# Autodesk Inventor assembly: EEZYbotARM Mk2
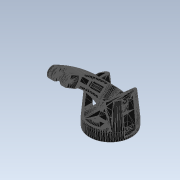
[picture p0: Inventor's stored thumbnail of the model, 180x180]
Saved by Autodesk Inventor 2022.5 (Build 265521000, 521)
## iProperties
Created: 2024-11-13
Part Number: EEZYbotARM Mk2
Document SubType Name: Assembly
Designer: Gagouking
Author: Gagouking
## Documents named in this file (3)
- D:\Documents\好玩的\水下机器人\EEZYbotARM Mk2.iam
- D:\Documents\RoboMaster\EBAmk2_001_base.ipt
- D:\Documents\RoboMaster\EBAmk2_002_mainarm.ipt
## Components (2 placed, 2 different names)
1. EBAmk2_001_base:1 — 配合:1, 配合:2
2. EBAmk2_002_mainarm:1 — 配合:1, 配合:2
## Relationships (2: Mate 2)
- 配合:1 [Mate]: EBAmk2_001_base:1 ↔ EBAmk2_002_mainarm:1
- 配合:2 [Mate]: EBAmk2_001_base:1 ↔ EBAmk2_002_mainarm:1
